# Autodesk Inventor assembly: Full Chassis with Arduino, Gyro, 1 inch Arms, and Konylak Wheels
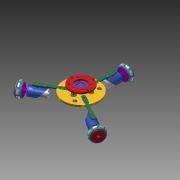
[picture p0: Inventor's stored thumbnail of the model, 180x180]
Saved by Autodesk Inventor 2014 (Build 180170000, 170)
## iProperties
Created: 2014-02-14
Part Number: Full Chassis with Arduino, Gyro, 1 inch Arms, and Konylak Wheels
Document SubType Name: Assembly
Designer: Spooner
Author: Spooner
## Documents named in this file (5)
- C:\Users\Spooner\Documents\Inventor\FerretBall Robot\3Pod\Inventor 2014 Files\Full Chassis with Arduino, Gyro, 1 inch Arms, and Konylak Wheels.iam
- C:\Users\Spooner\Documents\Inventor\FerretBall Robot\3Pod\Inventor 2014 Files\Main Body with Arduino and Gyro Mounts.iam
- C:\Users\Spooner\Documents\Inventor\Content Center Files\R2014\en-US\JIS B 1111(1)\JIS B 1111 - M3x10(1).ipt
- C:\Users\Spooner\Documents\Inventor\Content Center Files\R2014\en-US\JIS B 1181 U\JIS B 1181 - B M3.ipt
- C:\Users\Spooner\Documents\Inventor\FerretBall Robot\3Pod\Inventor 2014 Files\Full Motor Arm (1 inch) with Kornylak Wheel.iam
## Components (16 placed, 4 different names)
1. Main Body with Arduino and Gyro Mounts:1 [sub-assembly] — Insert:10, Insert:11, Insert:12, Insert:13, Insert:14, Insert:15, Insert:16, Insert:17, Insert:18
2. JIS B 1111 M3x10:1 — Insert:11, Mate:3
3. JIS B 1111 M3x10:2 — Insert:10
4. JIS B 1111 M3x10:3 — Insert:15, Mate:1
5. JIS B 1111 M3x10:4 — Insert:14
6. JIS B 1111 M3x10:5 — Insert:13, Mate:2
7. JIS B 1111 M3x10:6 — Insert:12
8. JIS B 1181 (unchamfered) - Metric B M3:1
9. JIS B 1181 (unchamfered) - Metric B M3:2
10. JIS B 1181 (unchamfered) - Metric B M3:3
11. JIS B 1181 (unchamfered) - Metric B M3:4
12. JIS B 1181 (unchamfered) - Metric B M3:5
13. JIS B 1181 (unchamfered) - Metric B M3:6
14. Full Motor Arm (1 inch) with Kornylak Wheel:1 [sub-assembly] — Insert:18, Mate:3
15. Full Motor Arm (1 inch) with Kornylak Wheel:2 [sub-assembly] — Insert:17, Mate:2
16. Full Motor Arm (1 inch) with Kornylak Wheel:3 [sub-assembly] — Insert:16, Mate:1
## Relationships (12: Insert 9, Mate 3)
- Insert:10: Main Body with Arduino and Gyro Mounts:1 ↔ JIS B 1111 M3x10:2
- Insert:11: Main Body with Arduino and Gyro Mounts:1 ↔ JIS B 1111 M3x10:1
- Insert:12: Main Body with Arduino and Gyro Mounts:1 ↔ JIS B 1111 M3x10:6
- Insert:13: Main Body with Arduino and Gyro Mounts:1 ↔ JIS B 1111 M3x10:5
- Insert:14: Main Body with Arduino and Gyro Mounts:1 ↔ JIS B 1111 M3x10:4
- Insert:15: Main Body with Arduino and Gyro Mounts:1 ↔ JIS B 1111 M3x10:3
- Insert:16: Main Body with Arduino and Gyro Mounts:1 ↔ Full Motor Arm (1 inch) with Kornylak Wheel:3
- Mate:1: JIS B 1111 M3x10:3 ↔ Full Motor Arm (1 inch) with Kornylak Wheel:3
- Insert:17: Main Body with Arduino and Gyro Mounts:1 ↔ Full Motor Arm (1 inch) with Kornylak Wheel:2
- Mate:2: JIS B 1111 M3x10:5 ↔ Full Motor Arm (1 inch) with Kornylak Wheel:2
- Insert:18: Main Body with Arduino and Gyro Mounts:1 ↔ Full Motor Arm (1 inch) with Kornylak Wheel:1
- Mate:3: JIS B 1111 M3x10:1 ↔ Full Motor Arm (1 inch) with Kornylak Wheel:1
